# Autodesk Inventor assembly: McCrea_final_scene_walle
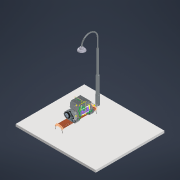
[picture p0: Inventor's stored thumbnail of the model, 180x180]
Saved by Autodesk Inventor 2022 (Build 260153000, 153)
## iProperties
Created: 2022-02-01
Part Number: McCrea_final_scene_walle
Document SubType Name: Assembly
Designer: MatusBarany
Author: MatusBarany
## Documents named in this file (5)
- C:\Users\MatusBarany\Documents\Inventor\wall-e\assembly\McCrea_final_scene_walle.iam
- C:\Users\MatusBarany\Documents\Inventor\wall-e\matus\plocha\McCrea_plocha_walle.ipt
- C:\Users\MatusBarany\Documents\Inventor\wall-e\matus\bench\McCrea_assembly_walle.iam
- C:\Users\MatusBarany\Documents\Inventor\wall-e\assembly\McCrea_WALLE_bez_HEAD_walle.iam
- C:\Users\MatusBarany\Documents\Inventor\wall-e\matus\lampa\McCrea_lampa_walle.ipt
## Components (4 placed, 4 different names)
1. McCrea_plocha_walle:1 — Mate:1, Mate:2
2. McCrea_assembly_walle:1 [sub-assembly] — Mate:1
3. McCrea_WALLE_bez_HEAD_walle:1 [sub-assembly]
4. McCrea_lampa_walle:1 — Mate:2
## Relationships (2: Mate 2)
- Mate:1: McCrea_plocha_walle:1 ↔ McCrea_assembly_walle:1
- Mate:2: McCrea_plocha_walle:1 ↔ McCrea_lampa_walle:1
